# Autodesk Inventor assembly: PrototypingShooterHalfFrame
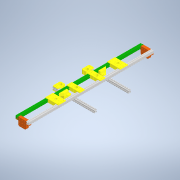
[picture p0: Inventor's stored thumbnail of the model, 180x180]
Saved by Autodesk Inventor 2020 (Build 240168000, 168)
## iProperties
Created: 2020-01-08
Part Number: PrototypingShooterHalfFrame
Document SubType Name: Assembly
Designer: srini
Author: srini
## Documents named in this file (9)
- C:\Users\srini\Documents\FRC\2020\PrototypingShooterHalfFrame.iam
- C:\Users\srini\Documents\FRC\2020\1003-48-CL.ipt
- C:\Users\srini\Documents\FRC\2020\9inSpacer.ipt
- C:\Users\srini\Documents\FRC\2020\90DegJoiner.ipt
- C:\Users\srini\Documents\FRC\2020\90DegJoiner_MIR.ipt
- C:\Users\srini\Documents\FRC\2020\CIMmount.ipt
- C:\Users\srini\Documents\FRC\2020\BearingMount.ipt
- C:\Users\srini\Documents\FRC\2020\1010-16-CL.ipt
- C:\Users\srini\Documents\FRC\2020\SingleSideBearing.ipt
## Components (14 placed, 8 different names)
1. 1003-48-CL:1 — Mate:1, Flush:1, Flush:2, Mate:2, Mate:3, Mate:4, Mate:5, Mate:6, Mate:7, Mate:8, Mate:9, Mate:10, Mate:11, Flush:3, Mate:12, Mate:13, Flush:4, Mate:14, Mate:15, Mate:16, Mate:17, Mate:19, Mate:20
2. 1003-48-CL:2 — Mate:1, Flush:1, Flush:2
3. 9inSpacer:1 — Mate:10, Mate:11, Flush:3
4. 9inSpacer:2 — Mate:12, Mate:13, Flush:4
5. 90DegJoiner:1 — Mate:14, Mate:15, Mate:18
6. 90DegJoiner_MIR:1 — Mate:16, Mate:17, Mate:21
7. CIMmount:1 — Mate:2, Mate:9
8. CIMmount:2 — Mate:3, Mate:6
9. BearingMount:1 — Mate:4, Mate:7
10. BearingMount:2 — Mate:5, Mate:8
11. 1010-16-CL:1 — Mate:18, Mate:19, Flush:5, Mate:22, Flush:6, Mate:23
12. 1010-16-CL:2 — Mate:20, Mate:21, Flush:5, Mate:24, Mate:25, Flush:7
13. SingleSideBearing:1 — Mate:22, Flush:6, Mate:23
14. SingleSideBearing:2 — Mate:24, Mate:25, Flush:7
## Relationships (32: Mate 25, Flush 7)
- Mate:1 (76.2 mm): 1003-48-CL:1 ↔ 1003-48-CL:2
- Flush:1: 1003-48-CL:1 ↔ 1003-48-CL:2
- Flush:2: 1003-48-CL:1 ↔ 1003-48-CL:2
- Mate:2: 1003-48-CL:1 ↔ CIMmount:1
- Mate:3: 1003-48-CL:1 ↔ CIMmount:2
- Mate:4: 1003-48-CL:1 ↔ BearingMount:1
- Mate:5: 1003-48-CL:1 ↔ BearingMount:2
- Mate:6: 1003-48-CL:1 ↔ CIMmount:2
- Mate:7: 1003-48-CL:1 ↔ BearingMount:1
- Mate:8: 1003-48-CL:1 ↔ BearingMount:2
- Mate:9: 1003-48-CL:1 ↔ CIMmount:1
- Mate:10: 1003-48-CL:1 ↔ 9inSpacer:1
- Mate:11: 1003-48-CL:1 ↔ 9inSpacer:1
- Flush:3: 1003-48-CL:1 ↔ 9inSpacer:1
- Mate:12: 1003-48-CL:1 ↔ 9inSpacer:2
- Mate:13: 1003-48-CL:1 ↔ 9inSpacer:2
- Flush:4: 1003-48-CL:1 ↔ 9inSpacer:2
- Mate:14: 1003-48-CL:1 ↔ 90DegJoiner:1
- Mate:15: 1003-48-CL:1 ↔ 90DegJoiner:1
- Mate:16: 1003-48-CL:1 ↔ 90DegJoiner_MIR:1
- Mate:17: 1003-48-CL:1 ↔ 90DegJoiner_MIR:1
- Mate:18: 90DegJoiner:1 ↔ 1010-16-CL:1
- Mate:19: 1003-48-CL:1 ↔ 1010-16-CL:1
- Mate:20: 1003-48-CL:1 ↔ 1010-16-CL:2
- Mate:21: 90DegJoiner_MIR:1 ↔ 1010-16-CL:2
- Flush:5: 1010-16-CL:1 ↔ 1010-16-CL:2
- Mate:22: 1010-16-CL:1 ↔ SingleSideBearing:1
- Flush:6: 1010-16-CL:1 ↔ SingleSideBearing:1
- Mate:23: 1010-16-CL:1 ↔ SingleSideBearing:1
- Mate:24: 1010-16-CL:2 ↔ SingleSideBearing:2
- Mate:25: 1010-16-CL:2 ↔ SingleSideBearing:2
- Flush:7: 1010-16-CL:2 ↔ SingleSideBearing:2
